# Autodesk Inventor assembly: Bed Plate Assembly
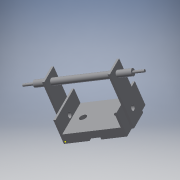
[picture p0: Inventor's stored thumbnail of the model, 180x180]
Saved by Autodesk Inventor 2018 (Build 220112000, 112)
## iProperties
Created: 2017-04-14
Part Number: Bed Plate Assembly
Document SubType Name: Assembly
Designer: Administrator
Author: Administrator
## Documents named in this file (5)
- C:\Users\Administrator\Documents\TA202\Bed Plate Assembly.iam
- C:\Users\Administrator\Documents\TA202\Bed Plate Support.ipt
- C:\Users\Administrator\Documents\TA202\Bed Plate.ipt
- C:\Users\Administrator\Documents\TA202\Bed Plate Hang.ipt
- C:\Users\Administrator\Documents\TA202\Bed Plate Axle.ipt
## Components (6 placed, 4 different names)
1. Bed Plate Support:1 — Mate:1, Mate:2, Flush:1, Mate:5, Mate:6, Angle:1
2. Bed Plate:1 — Mate:1, Mate:2, Flush:1, Flush:2, Mate:3, Mate:4
3. Bed Plate Support:2 — Flush:2, Mate:3, Mate:4, Mate:7, Angle:2, Mate:8
4. Bed Plate Hang:1 — Mate:5, Mate:6, Angle:1, Insert:1
5. Bed Plate Hang:2 — Mate:7, Angle:2, Mate:8
6. Bed Plate Axle:1 — Insert:1
## Relationships (13: Mate 8, Flush 2, Angle 2, Insert 1)
- Mate:1: Bed Plate Support:1 ↔ Bed Plate:1
- Mate:2: Bed Plate Support:1 ↔ Bed Plate:1
- Flush:1: Bed Plate Support:1 ↔ Bed Plate:1
- Flush:2: Bed Plate:1 ↔ Bed Plate Support:2
- Mate:3: Bed Plate:1 ↔ Bed Plate Support:2
- Mate:4: Bed Plate:1 ↔ Bed Plate Support:2
- Mate:5: Bed Plate Support:1 ↔ Bed Plate Hang:1
- Mate:6: Bed Plate Support:1 ↔ Bed Plate Hang:1
- Angle:1 (0 deg): Bed Plate Support:1 ↔ Bed Plate Hang:1
- Mate:7: Bed Plate Support:2 ↔ Bed Plate Hang:2
- Angle:2 (0 deg): Bed Plate Support:2 ↔ Bed Plate Hang:2
- Mate:8: Bed Plate Support:2 ↔ Bed Plate Hang:2
- Insert:1 (-15 mm): Bed Plate Hang:1 ↔ Bed Plate Axle:1
